# Autodesk Inventor assembly: SoapAssembly
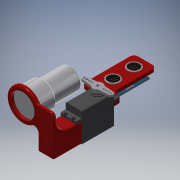
[picture p0: Inventor's stored thumbnail of the model, 180x180]
Saved by Autodesk Inventor 2018.3 (Build 223284000, 284)
## iProperties
Created: 2020-03-24
Part Number: SoapAssembly
Document SubType Name: Assembly
Designer: Ivan
Author: Ivan
## Documents named in this file (7)
- C:\Users\Ivan\Documents\GitHub\Soap-dispenser\3D Model\SoapAssembly.iam
- C:\Users\Ivan\Documents\GitHub\Soap-dispenser\3D Model\ServoSupport.ipt
- C:\Users\Ivan\Documents\GitHub\Soap-dispenser\3D Model\Servo MG995.ipt
- C:\Users\Ivan\Documents\GitHub\Soap-dispenser\3D Model\DispenserHead.ipt
- C:\Users\Ivan\Documents\GitHub\Soap-dispenser\3D Model\ServoArm2.ipt
- C:\Users\Ivan\Documents\GitHub\Soap-dispenser\3D Model\HC-SR04.ipt
- C:\Users\Ivan\Documents\GitHub\Soap-dispenser\3D Model\UltrasonicBase.ipt
## Components (6 placed, 6 different names)
1. ServoSupport:1 — Mate:1, Flush:1, Mate:2, Mate:3, Mate:4
2. Servo MG995:1 — Mate:1, Flush:1, Mate:2, Insert:1, Mate:5, Flush:2, Mate:6, Angle:1
3. DispenserHead:1 — Mate:3, Mate:4
4. ServoArm2:1 — Insert:1
5. HC-SR04:1 — Angle:1, Mate:7, Mate:8
6. UltrasonicBase:1 — Mate:5, Flush:2, Mate:6, Mate:7, Mate:8
## Relationships (12: Mate 8, Flush 2, Insert 1, Angle 1)
- Mate:1: ServoSupport:1 ↔ Servo MG995:1
- Flush:1: ServoSupport:1 ↔ Servo MG995:1
- Mate:2: ServoSupport:1 ↔ Servo MG995:1
- Mate:3: ServoSupport:1 ↔ DispenserHead:1
- Mate:4: ServoSupport:1 ↔ DispenserHead:1
- Insert:1: Servo MG995:1 ↔ ServoArm2:1
- Mate:5: Servo MG995:1 ↔ UltrasonicBase:1
- Flush:2: Servo MG995:1 ↔ UltrasonicBase:1
- Mate:6: Servo MG995:1 ↔ UltrasonicBase:1
- Angle:1 (0 deg): Servo MG995:1 ↔ HC-SR04:1
- Mate:7: HC-SR04:1 ↔ UltrasonicBase:1
- Mate:8: HC-SR04:1 ↔ UltrasonicBase:1
